# Autodesk Inventor assembly: extruder_mirrored
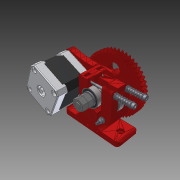
[picture p0: Inventor's stored thumbnail of the model, 180x180]
Saved by Autodesk Inventor 2014 (Build 180170000, 170)
## iProperties
Created: 2014-02-23
Part Number: extruder_mirrored
Document SubType Name: Assembly
Designer: buben
Author: buben
## Documents named in this file (17)
- C:\Users\buben\Documents\GitHub\bacon\inventor files\assemblies\extruder_mirrored.iam
- C:\Users\buben\Documents\GitHub\bacon\inventor files\3rd party components\gregs wade\jonaskuehling_gregs-wade-v3_jhead-BODY-ONLY_mirror.ipt
- C:\Users\buben\Documents\GitHub\bacon\inventor files\3rd party components\nema_17_stepper\Imported Components\NEMA 17\NEMA 17.iam
- C:\Users\buben\Documents\GitHub\bacon\inventor files\3rd party components\gregs wade\smallgearmod_fixed.ipt
- C:\Users\buben\Documents\GitHub\bacon\inventor files\3rd party components\gregs wade\biggearmod_fixed.ipt
- C:\Users\buben\Documents\GitHub\bacon\inventor files\3rd party components\gregs wade\jonaskuehling_gregs-wade-v3_idler-only.ipt
- C:\Users\buben\Documents\Inventor\Content Center Files\R2014\en-US\CSN EN 24014\ISO 4014 - M8 x 55CSN EN.ipt
- C:\Users\buben\Documents\GitHub\bacon\inventor files\utils\washer_m8.ipt
- C:\Users\buben\Documents\GitHub\bacon\inventor files\3rd party components\bearing_608\Imported Components\608RS\608RS.ipt
- C:\Users\buben\Documents\GitHub\bacon\inventor files\utils\extruder_bearing_shaft.ipt
- C:\Users\buben\Documents\Inventor\Content Center Files\R2014\en-US\ANSI B18.3.1M(6)\ANSI B18.3.1M - M3x0,5 x 35(1).ipt
- C:\Users\buben\Documents\GitHub\bacon\inventor files\utils\washer_m3.ipt
- C:\Users\buben\Documents\Inventor\Content Center Files\R2014\en-US\ISO 7040\ISO 7040 - M3.ipt
- C:\Users\buben\Documents\Inventor\Content Center Files\R2014\en-US\CSN EN 24032\ISO 4032 - M8CSN EN.ipt
- C:\Users\buben\Documents\Inventor\Content Center Files\R2014\en-US\ISO 4762(2)\ISO 4762 - M3 x 10ISO.ipt
- C:\Users\buben\Documents\GitHub\bacon\inventor files\assemblies\extruder\Design Accelerator\Compress Spring2.iam
- C:\Users\buben\Documents\Inventor\Content Center Files\R2014\en-US\ANSI B18.3.1M(6)\ANSI B18.3.1M - M3x0,5 x 60(1).ipt
## Components (34 placed, 16 different names)
1. jonaskuehling_gregs-wade-v3_jhead-BODY-ONLY_mirror:1 — Mate:1, Mate:2, Flush:1, Tangent:9, Tangent:10, Mate:18, Mate:19, Mate:21, Tangent:13, Tangent:14, Mate:28, Tangent:15, Tangent:16, Mate:38, Mate:39, Mate:40, Angle:2
2. NEMA 17:1 [sub-assembly] — Tangent:1, Tangent:2, Mate:21, Tangent:15, Tangent:16, Mate:35, Mate:36, Mate:37
3. smallgearmod_fixed:1 — Tangent:1, Tangent:2, Mate:22
4. biggearmod_fixed:1 — Tangent:3, Tangent:4, Angle:1, Mate:3, Mate:9, Mate:22
5. jonaskuehling_gregs-wade-v3_idler-only:1 — Tangent:7, Tangent:8, Mate:16, Mate:17, Mate:23, Mate:24, Tangent:11, Tangent:12, Mate:28, Mate:49, Mate:50, Tangent:17, Tangent:18, Tangent:19, Tangent:20, Angle:2
6. CSN EN 24014 M8 x 55:1 — Tangent:3, Tangent:4, Angle:1, Mate:3, Mate:8, Mate:10, Mate:20, Mate:30, Mate:33
7. CSN 02 1702 B B 8,4:1 — Mate:4, Mate:5, Mate:6, Mate:7
8. CSN 02 1702 B B 8,4:2 — Mate:5, Mate:6, Mate:8, Mate:9
9. CSN 02 1702 B B 8,4:3 — Mate:4, Mate:7, Mate:11
10. 608RS:2 — Mate:10, Mate:11, Mate:19
11. 608RS:3 — Mate:15, Mate:17
12. extruder_bearing_shaft:1 — Mate:15, Tangent:7, Tangent:8, Mate:16
13. 608RS:4 — Tangent:9, Tangent:10, Mate:18, Mate:20, Mate:29
14. Forged Socket Head Cap Screw - Metric M3x0,5 x 35:1 — Insert:1, Tangent:11, Tangent:12, Mate:25, Mate:27, Tangent:13, Tangent:14
15. CSN 02 1702 B B 3,2:1 — Mate:23, Mate:25, Mate:26
16. CSN 02 1702 B B 3,2:2 — Mate:24, Insert:1
17. DIN EN ISO 7040 M3:1 — Mate:26, Mate:27
18. CSN 02 1702 B B 8,4:4 — Mate:29, Mate:30, Mate:34
19. CSN EN 24032 M8:1 — Mate:31, Flush:2, Mate:32
20. CSN EN 24032 M8:2 — Mate:31, Flush:2, Mate:32, Mate:33, Mate:34
21. ISO 4762 M3 x 10:1 — Insert:2, Mate:36
22. ISO 4762 M3 x 10:2 — Insert:4, Mate:35
23. ISO 4762 M3 x 10:3 — Insert:3, Mate:37
24. CSN 02 1702 B B 3,2:3 — Insert:2, Mate:38
25. CSN 02 1702 B B 3,2:4 — Insert:3, Mate:40
26. CSN 02 1702 B B 3,2:5 — Insert:4, Mate:39
27. CSN 02 1702 B B 3,2:6 — Mate:50
28. Compress Spring:1 [sub-assembly]
29. CSN 02 1702 B B 3,2:7
30. Forged Socket Head Cap Screw - Metric M3x0,5 x 60:1 — Tangent:19, Tangent:20
31. CSN 02 1702 B B 3,2:8 — Mate:49
32. Compress Spring:2 [sub-assembly]
33. CSN 02 1702 B B 3,2:9
34. Forged Socket Head Cap Screw - Metric M3x0,5 x 60:2 — Tangent:17, Tangent:18
## Relationships (75: Mate 47, Tangent 18, Insert 6, Flush 2, Angle 2)
- Mate:1: jonaskuehling_gregs-wade-v3_jhead-BODY-ONLY_mirror:1
- Mate:2: jonaskuehling_gregs-wade-v3_jhead-BODY-ONLY_mirror:1
- Flush:1: jonaskuehling_gregs-wade-v3_jhead-BODY-ONLY_mirror:1
- Tangent:1: NEMA 17:1 ↔ smallgearmod_fixed:1
- Tangent:2: NEMA 17:1 ↔ smallgearmod_fixed:1
- Tangent:3 (0.2 mm): biggearmod_fixed:1 ↔ CSN EN 24014 M8 x 55:1
- Tangent:4 (0.2 mm): biggearmod_fixed:1 ↔ CSN EN 24014 M8 x 55:1
- Angle:1 (0 deg): biggearmod_fixed:1 ↔ CSN EN 24014 M8 x 55:1
- Mate:3: biggearmod_fixed:1 ↔ CSN EN 24014 M8 x 55:1
- Mate:4: CSN 02 1702 B B 8,4:1 ↔ CSN 02 1702 B B 8,4:3
- Mate:5: CSN 02 1702 B B 8,4:1 ↔ CSN 02 1702 B B 8,4:2
- Mate:6: CSN 02 1702 B B 8,4:1 ↔ CSN 02 1702 B B 8,4:2
- Mate:7: CSN 02 1702 B B 8,4:1 ↔ CSN 02 1702 B B 8,4:3
- Mate:8: CSN EN 24014 M8 x 55:1 ↔ CSN 02 1702 B B 8,4:2
- Mate:9: biggearmod_fixed:1 ↔ CSN 02 1702 B B 8,4:2
- Mate:10: CSN EN 24014 M8 x 55:1 ↔ 608RS:2
- Mate:11: CSN 02 1702 B B 8,4:3 ↔ 608RS:2
- Mate:15: 608RS:3 ↔ extruder_bearing_shaft:1
- Tangent:7: jonaskuehling_gregs-wade-v3_idler-only:1 ↔ extruder_bearing_shaft:1
- Tangent:8: jonaskuehling_gregs-wade-v3_idler-only:1 ↔ extruder_bearing_shaft:1
- Mate:16: jonaskuehling_gregs-wade-v3_idler-only:1 ↔ extruder_bearing_shaft:1
- Mate:17: jonaskuehling_gregs-wade-v3_idler-only:1 ↔ 608RS:3
- Tangent:9 (0.2 mm): jonaskuehling_gregs-wade-v3_jhead-BODY-ONLY_mirror:1 ↔ 608RS:4
- Tangent:10 (0.2 mm): jonaskuehling_gregs-wade-v3_jhead-BODY-ONLY_mirror:1 ↔ 608RS:4
- Mate:18: jonaskuehling_gregs-wade-v3_jhead-BODY-ONLY_mirror:1 ↔ 608RS:4
- Mate:19: jonaskuehling_gregs-wade-v3_jhead-BODY-ONLY_mirror:1 ↔ 608RS:2
- Mate:20: CSN EN 24014 M8 x 55:1 ↔ 608RS:4
- Mate:21: jonaskuehling_gregs-wade-v3_jhead-BODY-ONLY_mirror:1 ↔ NEMA 17:1
- Mate:22 (0.75 mm): smallgearmod_fixed:1 ↔ biggearmod_fixed:1
- Mate:23: jonaskuehling_gregs-wade-v3_idler-only:1 ↔ CSN 02 1702 B B 3,2:1
- Mate:24: jonaskuehling_gregs-wade-v3_idler-only:1 ↔ CSN 02 1702 B B 3,2:2
- Insert:1: Forged Socket Head Cap Screw - Metric M3x0,5 x 35:1 ↔ CSN 02 1702 B B 3,2:2
- Tangent:11: jonaskuehling_gregs-wade-v3_idler-only:1 ↔ Forged Socket Head Cap Screw - Metric M3x0,5 x 35:1
- Tangent:12: jonaskuehling_gregs-wade-v3_idler-only:1 ↔ Forged Socket Head Cap Screw - Metric M3x0,5 x 35:1
- Mate:25: Forged Socket Head Cap Screw - Metric M3x0,5 x 35:1 ↔ CSN 02 1702 B B 3,2:1
- Mate:26: CSN 02 1702 B B 3,2:1 ↔ DIN EN ISO 7040 M3:1
- Mate:27: Forged Socket Head Cap Screw - Metric M3x0,5 x 35:1 ↔ DIN EN ISO 7040 M3:1
- Tangent:13: jonaskuehling_gregs-wade-v3_jhead-BODY-ONLY_mirror:1 ↔ Forged Socket Head Cap Screw - Metric M3x0,5 x 35:1
- Tangent:14: jonaskuehling_gregs-wade-v3_jhead-BODY-ONLY_mirror:1 ↔ Forged Socket Head Cap Screw - Metric M3x0,5 x 35:1
- Mate:28: jonaskuehling_gregs-wade-v3_jhead-BODY-ONLY_mirror:1 ↔ jonaskuehling_gregs-wade-v3_idler-only:1
- Mate:29: 608RS:4 ↔ CSN 02 1702 B B 8,4:4
- Mate:30: CSN EN 24014 M8 x 55:1 ↔ CSN 02 1702 B B 8,4:4
- Mate:31: CSN EN 24032 M8:1 ↔ CSN EN 24032 M8:2
- Flush:2: CSN EN 24032 M8:1 ↔ CSN EN 24032 M8:2
- Mate:32: CSN EN 24032 M8:1 ↔ CSN EN 24032 M8:2
- Mate:33: CSN EN 24014 M8 x 55:1 ↔ CSN EN 24032 M8:2
- Mate:34: CSN 02 1702 B B 8,4:4 ↔ CSN EN 24032 M8:2
- Tangent:15 (0.5 mm): jonaskuehling_gregs-wade-v3_jhead-BODY-ONLY_mirror:1 ↔ NEMA 17:1
- Tangent:16 (0.5 mm): jonaskuehling_gregs-wade-v3_jhead-BODY-ONLY_mirror:1 ↔ NEMA 17:1
- Insert:2: ISO 4762 M3 x 10:1 ↔ CSN 02 1702 B B 3,2:3
- Insert:3: ISO 4762 M3 x 10:3 ↔ CSN 02 1702 B B 3,2:4
- Insert:4: ISO 4762 M3 x 10:2 ↔ CSN 02 1702 B B 3,2:5
- Mate:35: NEMA 17:1 ↔ ISO 4762 M3 x 10:2
- Mate:36: NEMA 17:1 ↔ ISO 4762 M3 x 10:1
- Mate:37: NEMA 17:1 ↔ ISO 4762 M3 x 10:3
- Mate:38: jonaskuehling_gregs-wade-v3_jhead-BODY-ONLY_mirror:1 ↔ CSN 02 1702 B B 3,2:3
- Mate:39: jonaskuehling_gregs-wade-v3_jhead-BODY-ONLY_mirror:1 ↔ CSN 02 1702 B B 3,2:5
- Mate:40: jonaskuehling_gregs-wade-v3_jhead-BODY-ONLY_mirror:1 ↔ CSN 02 1702 B B 3,2:4
- [Mate]: CSN 02 1702 B B 3,2:6 ↔ Compress Spring:1
- [Mate]: CSN 02 1702 B B 3,2:6 ↔ Compress Spring:1
- [Mate]: Compress Spring:1 ↔ CSN 02 1702 B B 3,2:7
- [Mate]: CSN 02 1702 B B 3,2:6 ↔ CSN 02 1702 B B 3,2:7
- [Insert]: CSN 02 1702 B B 3,2:7 ↔ Forged Socket Head Cap Screw - Metric M3x0,5 x 60:1
- [Mate]: CSN 02 1702 B B 3,2:8 ↔ Compress Spring:2
- [Mate]: CSN 02 1702 B B 3,2:8 ↔ Compress Spring:2
- [Mate]: Compress Spring:2 ↔ CSN 02 1702 B B 3,2:9
- [Mate]: CSN 02 1702 B B 3,2:8 ↔ CSN 02 1702 B B 3,2:9
- [Insert]: CSN 02 1702 B B 3,2:9 ↔ Forged Socket Head Cap Screw - Metric M3x0,5 x 60:2
- Mate:49: jonaskuehling_gregs-wade-v3_idler-only:1 ↔ CSN 02 1702 B B 3,2:8
- Mate:50: jonaskuehling_gregs-wade-v3_idler-only:1 ↔ CSN 02 1702 B B 3,2:6
- Tangent:17 (1 mm): jonaskuehling_gregs-wade-v3_idler-only:1 ↔ Forged Socket Head Cap Screw - Metric M3x0,5 x 60:2
- Tangent:18 (1 mm): jonaskuehling_gregs-wade-v3_idler-only:1 ↔ Forged Socket Head Cap Screw - Metric M3x0,5 x 60:2
- Tangent:19 (1 mm): jonaskuehling_gregs-wade-v3_idler-only:1 ↔ Forged Socket Head Cap Screw - Metric M3x0,5 x 60:1
- Tangent:20 (1 mm): jonaskuehling_gregs-wade-v3_idler-only:1 ↔ Forged Socket Head Cap Screw - Metric M3x0,5 x 60:1
- Angle:2 (0 deg): jonaskuehling_gregs-wade-v3_jhead-BODY-ONLY_mirror:1 ↔ jonaskuehling_gregs-wade-v3_idler-only:1
## Named parameters: d63_d64 = 0 mm, d64_d65 = 0 mm, d65_d66 = 0 mm, d66_d67 = 0 mm, d73_d70 = 0 mm
